# Autodesk Inventor assembly: maze_prototip
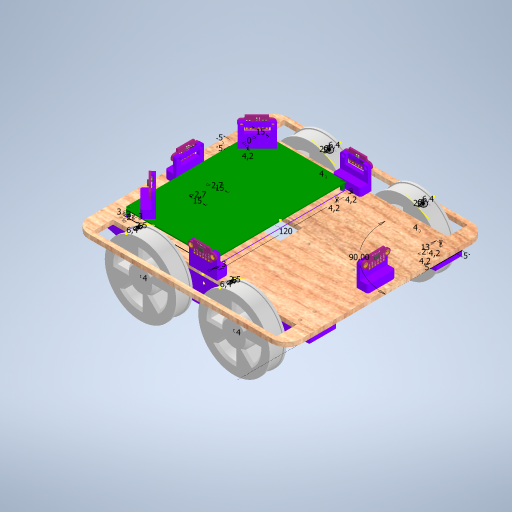
[picture p0: Inventor's stored thumbnail of the model, 512x512]
Saved by Autodesk Inventor 2023 (Build 270158000, 158)
## iProperties
Created: 2025-12-14
Part Number: maze_prototip
Document SubType Name: Assembly
Designer: garin
Author: garin
## Documents named in this file (11)
- C:\Users\garin\OneDrive\Документы\maze\prototip\maze_prototip.iam
- C:\Users\garin\OneDrive\Документы\maze\prototip\основа.ipt
- C:\Users\garin\OneDrive\Документы\maze\prototip\крепёж_для_мотора.ipt
- C:\Users\garin\OneDrive\Документы\maze\prototip\макетная плата.ipt
- C:\Users\garin\OneDrive\Документы\maze\prototip\крепление_RGB.ipt
- C:\Users\garin\OneDrive\Документы\maze\prototip\крепл_ЛД.ipt
- C:\Users\garin\OneDrive\Документы\Good morning 25 dc motor.ipt
- C:\Users\garin\OneDrive\Документы\maze\prototip\колеса прототип.ipt
- C:\Users\garin\OneDrive\Документы\COUPLE FLANGE.ipt
- C:\Users\garin\OneDrive\Документы\VL53L0X_TOF.ipt
- C:\Users\garin\OneDrive\Документы\TCS34725 RGB sensor.ipt
## Components (30 placed, 10 different names)
1. основа:1 — С поворотом:1, С поворотом:2, Заподлицо:1, С поворотом:3, Жесткий:1, Жесткий:2, С поворотом:4, С поворотом:5
2. крепёж_для_мотора:1 — С поворотом:1, С поворотом:9, С поворотом:11, С поворотом:14, С поворотом:15
3. крепёж_для_мотора:2 — С поворотом:2, С поворотом:8, С поворотом:10, С поворотом:12, С поворотом:13
4. макетная плата:1 — Заподлицо:1, С поворотом:6, С поворотом:7
5. крепление_RGB:1 — С поворотом:3, С поворотом:26
6. крепл_ЛД:1 — Жесткий:1, С поворотом:20
7. крепл_ЛД:2 — Жесткий:2, С поворотом:24
8. крепл_ЛД:3 — С поворотом:4, С поворотом:25
9. крепл_ЛД:4 — С поворотом:5, С поворотом:23
10. крепл_ЛД:5 — С поворотом:6, С поворотом:21
11. крепл_ЛД:6 — С поворотом:7, С поворотом:22
12. Good morning 25 dc motor:1 — С поворотом:8
13. Good morning 25 dc motor:2 — С поворотом:9
14. Good morning 25 dc motor:3 — С поворотом:10
15. Good morning 25 dc motor:4 — С поворотом:11
16. COUPLE FLANGE:1 — С поворотом:13, С поворотом:17
17. COUPLE FLANGE:2 — С поворотом:14, С поворотом:18
18. COUPLE FLANGE:3 — С поворотом:12, С поворотом:16
19. COUPLE FLANGE:4 — С поворотом:15, С поворотом:19
20. колеса прототип:1 — С поворотом:16
21. колеса прототип:2 — С поворотом:17
22. колеса прототип:3 — С поворотом:18
23. колеса прототип:4 — С поворотом:19
24. VL53L0X_TOF:1 — С поворотом:20
25. VL53L0X_TOF:2 — С поворотом:21
26. VL53L0X_TOF:3 — С поворотом:22
27. VL53L0X_TOF:4 — С поворотом:23
28. VL53L0X_TOF:5 — С поворотом:24
29. VL53L0X_TOF:6 — С поворотом:25
30. TCS34725 RGB sensor:1 — С поворотом:26
## Relationships (29: RevoluteJoint 26, WeldJoint 2, Flush 1)
- С поворотом:1 [RevoluteJoint]: основа:1 ↔ крепёж_для_мотора:1
- С поворотом:2 [RevoluteJoint]: основа:1 ↔ крепёж_для_мотора:2
- Заподлицо:1 [Flush]: основа:1 ↔ макетная плата:1
- С поворотом:3 [RevoluteJoint]: основа:1 ↔ крепление_RGB:1
- Жесткий:1 [WeldJoint]: основа:1 ↔ крепл_ЛД:1
- Жесткий:2 [WeldJoint]: основа:1 ↔ крепл_ЛД:2
- С поворотом:4 [RevoluteJoint]: основа:1 ↔ крепл_ЛД:3
- С поворотом:5 [RevoluteJoint]: основа:1 ↔ крепл_ЛД:4
- С поворотом:6 [RevoluteJoint]: макетная плата:1 ↔ крепл_ЛД:5
- С поворотом:7 [RevoluteJoint]: макетная плата:1 ↔ крепл_ЛД:6
- С поворотом:8 [RevoluteJoint]: крепёж_для_мотора:2 ↔ Good morning 25 dc motor:1
- С поворотом:9 [RevoluteJoint]: крепёж_для_мотора:1 ↔ Good morning 25 dc motor:2
- С поворотом:10 [RevoluteJoint]: крепёж_для_мотора:2 ↔ Good morning 25 dc motor:3
- С поворотом:11 [RevoluteJoint]: крепёж_для_мотора:1 ↔ Good morning 25 dc motor:4
- С поворотом:12 [RevoluteJoint]: крепёж_для_мотора:2 ↔ COUPLE FLANGE:3
- С поворотом:13 [RevoluteJoint]: крепёж_для_мотора:2 ↔ COUPLE FLANGE:1
- С поворотом:14 [RevoluteJoint]: крепёж_для_мотора:1 ↔ COUPLE FLANGE:2
- С поворотом:15 [RevoluteJoint]: крепёж_для_мотора:1 ↔ COUPLE FLANGE:4
- С поворотом:16 [RevoluteJoint]: COUPLE FLANGE:3 ↔ колеса прототип:1
- С поворотом:17 [RevoluteJoint]: COUPLE FLANGE:1 ↔ колеса прототип:2
- С поворотом:18 [RevoluteJoint]: COUPLE FLANGE:2 ↔ колеса прототип:3
- С поворотом:19 [RevoluteJoint]: COUPLE FLANGE:4 ↔ колеса прототип:4
- С поворотом:20 [RevoluteJoint]: крепл_ЛД:1 ↔ VL53L0X_TOF:1
- С поворотом:21 [RevoluteJoint]: крепл_ЛД:5 ↔ VL53L0X_TOF:2
- С поворотом:22 [RevoluteJoint]: крепл_ЛД:6 ↔ VL53L0X_TOF:3
- С поворотом:23 [RevoluteJoint]: крепл_ЛД:4 ↔ VL53L0X_TOF:4
- С поворотом:24 [RevoluteJoint]: крепл_ЛД:2 ↔ VL53L0X_TOF:5
- С поворотом:25 [RevoluteJoint]: крепл_ЛД:3 ↔ VL53L0X_TOF:6
- С поворотом:26 [RevoluteJoint]: крепление_RGB:1 ↔ TCS34725 RGB sensor:1
